# Autodesk Inventor assembly: Assembly_1
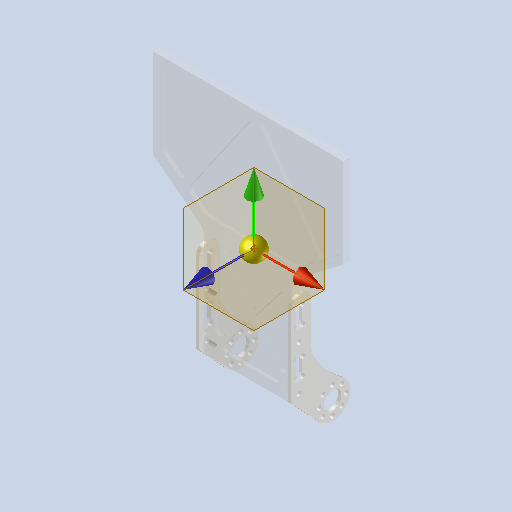
[picture p0: Inventor's stored thumbnail of the model, 512x512]
Saved by Autodesk Inventor 2024 (Build 280153000, 153)
## iProperties
Created: 2023-12-22
Part Number: Assembly_1
Document SubType Name: Assembly
Designer: right
Mass: 19.6823 g
Surface Area: 181.871 cm^2
Volume: 14.2057 cm^3
Density: 1.38551 g/cm^3
Author: right
## Documents named in this file (9)
- C:\Users\right\OneDrive\ドキュメント\Inventor\V2二足Light＿仮\Assembly_1.iam
- C:\Users\right\OneDrive\ドキュメント\Inventor\V2二足Light＿仮\tesaki_new.ipt
- C:\Users\right\OneDrive\ドキュメント\Inventor\V2二足Light＿仮\new_hera.ipt
- C:\Users\right\OneDrive\ドキュメント\Inventor\V2二足Light＿仮\Assembly_1\AIP\FEA\ek0kgxgf4.fins
- C:\Users\right\OneDrive\ドキュメント\Inventor\V2二足Light＿仮\Assembly_1\AIP\FEA\ek0kgxgkg.fsat
- C:\Users\right\OneDrive\ドキュメント\Inventor\V2二足Light＿仮\Assembly_1\AIP\FEA\ek0kgxgkg.ftes
- C:\Users\right\OneDrive\ドキュメント\Inventor\V2二足Light＿仮\Assembly_1\AIP\FEA\ek0kgxgkg.fwiz
- C:\Users\right\OneDrive\ドキュメント\Inventor\V2二足Light＿仮\Assembly_1\AIP\FEA\ek0kgxhfk.fmsh
- C:\Users\right\OneDrive\ドキュメント\Inventor\V2二足Light＿仮\Assembly_1\AIP\FEA\ek0kgxhgg.fres
## Components (3 placed, 2 different names)
1. tesaki_new:1
2. tesaki_new:2
3. new_hera:1
## Relationships (2: Insert 2)
- [Insert]: tesaki_new:2 ↔ new_hera:1
- [Insert]: tesaki_new:2 ↔ new_hera:1
## Named parameters: sa_0 = 0, sa_1 = 0, sa_2 = -980
note: some values were not read from the file. Shown as the stored number, unit unknown: "sa_0", "sa_1", "sa_2".
